# Autodesk Inventor assembly: Shooter Curve Assembly
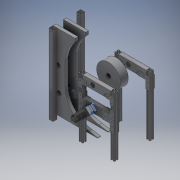
[picture p0: Inventor's stored thumbnail of the model, 180x180]
Saved by Autodesk Inventor 2018 (Build 220112000, 112)
## iProperties
Created: 2020-02-01
Part Number: Shooter Curve Assembly
Document SubType Name: Assembly
Designer: Weeb No1
Author: Weeb No1
## Documents named in this file (13)
- C:\Users\T3500STATIC\Documents\GitHub\2020CAD\Gabriel Inventor Files (Shooter, Drivebase)\V2 Shooter Curve Assembly\Main Assembly File\V2 Shooter Curve Assembly.iam
- C:\Users\T3500STATIC\Documents\GitHub\2020CAD\Gabriel Inventor Files (Shooter, Drivebase)\V2 Shooter Curve Assembly\Part Files\8020 1010 x 15.ipt
- C:\Users\T3500STATIC\Documents\GitHub\2020CAD\Gabriel Inventor Files (Shooter, Drivebase)\V2 Shooter Curve Assembly\Part Files\1x2 5 in Beam Flywheel Mount.ipt
- C:\Users\T3500STATIC\Documents\GitHub\2020CAD\Over bumper intake\Parts\VersaPlanetary_v2_Single_Stage_10_1_with_775_Series.iam
- C:\Users\T3500STATIC\Documents\GitHub\2020CAD\Gabriel Inventor Files (Shooter, Drivebase)\V2 Shooter Curve Assembly\Part Files\1x2 7 in Beam Motor Mount.ipt
- C:\Users\T3500STATIC\Documents\GitHub\2020CAD\Gabriel Inventor Files (Shooter, Drivebase)\Gussets\L-Gusset 3 Hole 0.25in Hole.ipt
- C:\Users\T3500STATIC\Documents\GitHub\2020CAD\Gabriel Inventor Files (Shooter, Drivebase)\V2 Shooter Curve Assembly\Part Files\1x1 20 in Curve Support Beam.ipt
- C:\Users\T3500STATIC\Documents\GitHub\2020CAD\Gabriel Inventor Files (Shooter, Drivebase)\Gussets\L-Guesset 4 Hole 0.25in Hole.ipt
- C:\Users\T3500STATIC\Documents\GitHub\2020CAD\Gabriel Inventor Files (Shooter, Drivebase)\Gussets\L-Guesset 5 Hole 0.25in Hole.ipt
- C:\Users\T3500STATIC\Documents\GitHub\2020CAD\Gabriel Inventor Files (Shooter, Drivebase)\V2 Shooter Curve Assembly\Part Files\_18t_Aluminum_Hub_Sprocket_25_Chain_1_2_Hex_Bore_217-3488.ipt
- C:\Users\T3500STATIC\Documents\GitHub\2020CAD\Gabriel Inventor Files (Shooter, Drivebase)\V2 Shooter Curve Assembly\Part Files\2_OD_Straight_Flex_Wheel_217-6354.ipt
- C:\Users\T3500STATIC\Documents\GitHub\2020CAD\Gabriel Inventor Files (Shooter, Drivebase)\V2 Shooter Curve Assembly\Part Files\New Shooter Curve.ipt
- C:\Users\T3500STATIC\Documents\GitHub\2020CAD\Gabriel Inventor Files (Shooter, Drivebase)\V2 Shooter Curve Assembly\Part Files\Pretend it's a Flywheel.ipt
## Components (33 placed, 12 different names)
1. 8020 1010 x 15:1 — Flush:5, Flush:6, Mate:7, Flush:11, Flush:14, Flush:23, Flush:24, Mate:51, Mate:56, Mate:60, Mate:82, Mate:85, Mate:97, Mate:100, Flush:45, Flush:48, Flush:52
2. 8020 1010 x 15:2 — Flush:7, Mate:9, Flush:15, Flush:22, Flush:25, Mate:127, Mate:130, Flush:44, Flush:46, Flush:51
3. 8020 1010 x 15:3 — Flush:5, Flush:6, Flush:10, Flush:12, Flush:13, Mate:11, Flush:23, Mate:50, Flush:34, Mate:63, Mate:65, Mate:89, Mate:93, Mate:103, Mate:123, Flush:49
4. 8020 1010 x 15:4 — Flush:7, Flush:10, Flush:17, Mate:10, Flush:22, Mate:107, Mate:111, Flush:47
5. 1x2 5 in Beam Flywheel Mount:1 — Mate:9, Flush:15, Flush:17, Mate:10, Flush:25, Mate:106, Mate:108, Mate:109, Mate:110, Mate:112, Mate:113, Mate:126, Mate:128, Mate:129, Mate:131, Mate:137, Flush:50, Mate:138, Mate:140
6. 1x2 5 in Beam Flywheel Mount:2 — Mate:7, Flush:11, Flush:12, Flush:13, Flush:14, Mate:11, Flush:24, Mate:55, Mate:57, Mate:58, Mate:59, Mate:61, Mate:62, Mate:64, Mate:66, Mate:137, Flush:50, Mate:139, Mate:141
7. VersaPlanetary_v2_Single_Stage_10_1_with_775_Series:1 [sub-assembly] — Mate:52, Mate:53, Mate:54
8. 1x2 7 in Beam Motor Mount:1 — Mate:50, Mate:51, Flush:34, Mate:52, Mate:53, Mate:54, Mate:81, Mate:83, Mate:86, Mate:87, Mate:88, Mate:90, Mate:91, Mate:92, Mate:94, Mate:95, Mate:96, Mate:98, Mate:99, Mate:101, Mate:102, Mate:104, Mate:105, Mate:122, Mate:124, Mate:125
9. L-Gusset 3 Hole 0.25in Hole:1 — Mate:61, Mate:62, Mate:63
10. L-Gusset 3 Hole 0.25in Hole:2 — Mate:55, Mate:56, Mate:57
11. L-Gusset 3 Hole 0.25in Hole:3 — Mate:58, Mate:59, Mate:60
12. L-Gusset 3 Hole 0.25in Hole:4 — Mate:64, Mate:65, Mate:66
13. 1x1 20 in Curve Support Beam:1 — Mate:132, Flush:35, Flush:36, Flush:40, Flush:41, Flush:45, Flush:52
14. 1x1 20 in Curve Support Beam:2 — Mate:133, Flush:37, Flush:38, Flush:39, Flush:41, Flush:44, Flush:51
15. L-Guesset 4 Hole 0.25in Hole:3 — Mate:88, Mate:89, Mate:90, Mate:91
16. L-Guesset 4 Hole 0.25in Hole:5 — Mate:81, Mate:82, Mate:83
17. L-Guesset 4 Hole 0.25in Hole:6 — Mate:85, Mate:86, Mate:87
18. L-Guesset 4 Hole 0.25in Hole:9 — Mate:92, Mate:93, Mate:94, Mate:95
19. L-Gusset 3 Hole 0.25in Hole:9 — Mate:96, Mate:97, Mate:98
20. L-Gusset 3 Hole 0.25in Hole:10 — Mate:99, Mate:100, Mate:101
21. L-Guesset 5 Hole 0.25in Hole:1 — Mate:102, Mate:103, Mate:104, Mate:105
22. L-Guesset 5 Hole 0.25in Hole:2 — Mate:110, Mate:111, Mate:112, Mate:113
23. L-Guesset 5 Hole 0.25in Hole:3 — Mate:106, Mate:107, Mate:108, Mate:109
24. L-Guesset 5 Hole 0.25in Hole:6 — Mate:122, Mate:123, Mate:124, Mate:125
25. L-Gusset 3 Hole 0.25in Hole:11 — Mate:126, Mate:127, Mate:128
26. L-Gusset 3 Hole 0.25in Hole:12 — Mate:129, Mate:130, Mate:131
27. _18t_Aluminum_Hub_Sprocket_25_Chain_1_2_Hex_Bore_217-3488:1
28. 2_OD_Straight_Flex_Wheel_217-6354:1
29. 2_OD_Straight_Flex_Wheel_217-6354:2
30. New Shooter Curve:1 — Mate:132, Flush:35, Flush:36, Flush:40, Mate:135, Mate:136, Flush:42, Flush:43, Flush:48, Flush:49, Flush:53, Flush:55
31. New Shooter Curve:2 — Mate:134, Mate:135, Flush:53, Flush:54, Flush:55, Flush:56
32. New Shooter Curve:3 — Mate:133, Flush:37, Flush:38, Flush:39, Mate:134, Mate:136, Flush:42, Flush:43, Flush:46, Flush:47, Flush:54, Flush:56
33. Pretend it's a Flywheel:1 — Mate:138, Mate:139, Mate:140, Mate:141
## Relationships (110: Mate 73, Flush 37)
- Flush:5: 8020 1010 x 15:1 ↔ 8020 1010 x 15:3
- Flush:6: 8020 1010 x 15:1 ↔ 8020 1010 x 15:3
- Flush:7: 8020 1010 x 15:2 ↔ 8020 1010 x 15:4
- Flush:10: 8020 1010 x 15:3 ↔ 8020 1010 x 15:4
- Mate:7: 8020 1010 x 15:1 ↔ 1x2 5 in Beam Flywheel Mount:2
- Flush:11: 8020 1010 x 15:1 ↔ 1x2 5 in Beam Flywheel Mount:2
- Flush:12: 8020 1010 x 15:3 ↔ 1x2 5 in Beam Flywheel Mount:2
- Flush:13: 8020 1010 x 15:3 ↔ 1x2 5 in Beam Flywheel Mount:2
- Flush:14: 8020 1010 x 15:1 ↔ 1x2 5 in Beam Flywheel Mount:2
- Mate:9: 8020 1010 x 15:2 ↔ 1x2 5 in Beam Flywheel Mount:1
- Flush:15: 8020 1010 x 15:2 ↔ 1x2 5 in Beam Flywheel Mount:1
- Flush:17: 8020 1010 x 15:4 ↔ 1x2 5 in Beam Flywheel Mount:1
- Mate:10: 8020 1010 x 15:4 ↔ 1x2 5 in Beam Flywheel Mount:1
- Mate:11: 8020 1010 x 15:3 ↔ 1x2 5 in Beam Flywheel Mount:2
- Flush:22: 8020 1010 x 15:2 ↔ 8020 1010 x 15:4
- Flush:23: 8020 1010 x 15:1 ↔ 8020 1010 x 15:3
- Flush:24: 8020 1010 x 15:1 ↔ 1x2 5 in Beam Flywheel Mount:2
- Flush:25: 8020 1010 x 15:2 ↔ 1x2 5 in Beam Flywheel Mount:1
- Mate:50: 8020 1010 x 15:3 ↔ 1x2 7 in Beam Motor Mount:1
- Mate:51: 8020 1010 x 15:1 ↔ 1x2 7 in Beam Motor Mount:1
- Flush:34: 8020 1010 x 15:3 ↔ 1x2 7 in Beam Motor Mount:1
- Mate:52: VersaPlanetary_v2_Single_Stage_10_1_with_775_Series:1 ↔ 1x2 7 in Beam Motor Mount:1
- Mate:53: VersaPlanetary_v2_Single_Stage_10_1_with_775_Series:1 ↔ 1x2 7 in Beam Motor Mount:1
- Mate:54: VersaPlanetary_v2_Single_Stage_10_1_with_775_Series:1 ↔ 1x2 7 in Beam Motor Mount:1
- Mate:55: 1x2 5 in Beam Flywheel Mount:2 ↔ L-Gusset 3 Hole 0.25in Hole:2
- Mate:56: 8020 1010 x 15:1 ↔ L-Gusset 3 Hole 0.25in Hole:2
- Mate:57: 1x2 5 in Beam Flywheel Mount:2 ↔ L-Gusset 3 Hole 0.25in Hole:2
- Mate:58: 1x2 5 in Beam Flywheel Mount:2 ↔ L-Gusset 3 Hole 0.25in Hole:3
- Mate:59: 1x2 5 in Beam Flywheel Mount:2 ↔ L-Gusset 3 Hole 0.25in Hole:3
- Mate:60: 8020 1010 x 15:1 ↔ L-Gusset 3 Hole 0.25in Hole:3
- Mate:61: 1x2 5 in Beam Flywheel Mount:2 ↔ L-Gusset 3 Hole 0.25in Hole:1
- Mate:62: 1x2 5 in Beam Flywheel Mount:2 ↔ L-Gusset 3 Hole 0.25in Hole:1
- Mate:63: 8020 1010 x 15:3 ↔ L-Gusset 3 Hole 0.25in Hole:1
- Mate:64: 1x2 5 in Beam Flywheel Mount:2 ↔ L-Gusset 3 Hole 0.25in Hole:4
- Mate:65: 8020 1010 x 15:3 ↔ L-Gusset 3 Hole 0.25in Hole:4
- Mate:66: 1x2 5 in Beam Flywheel Mount:2 ↔ L-Gusset 3 Hole 0.25in Hole:4
- Mate:81: 1x2 7 in Beam Motor Mount:1 ↔ L-Guesset 4 Hole 0.25in Hole:5
- Mate:82: 8020 1010 x 15:1 ↔ L-Guesset 4 Hole 0.25in Hole:5
- Mate:83: 1x2 7 in Beam Motor Mount:1 ↔ L-Guesset 4 Hole 0.25in Hole:5
- Mate:85: 8020 1010 x 15:1 ↔ L-Guesset 4 Hole 0.25in Hole:6
- Mate:86: 1x2 7 in Beam Motor Mount:1 ↔ L-Guesset 4 Hole 0.25in Hole:6
- Mate:87: 1x2 7 in Beam Motor Mount:1 ↔ L-Guesset 4 Hole 0.25in Hole:6
- Mate:88: 1x2 7 in Beam Motor Mount:1 ↔ L-Guesset 4 Hole 0.25in Hole:3
- Mate:89: 8020 1010 x 15:3 ↔ L-Guesset 4 Hole 0.25in Hole:3
- Mate:90: 1x2 7 in Beam Motor Mount:1 ↔ L-Guesset 4 Hole 0.25in Hole:3
- Mate:91: 1x2 7 in Beam Motor Mount:1 ↔ L-Guesset 4 Hole 0.25in Hole:3
- Mate:92: 1x2 7 in Beam Motor Mount:1 ↔ L-Guesset 4 Hole 0.25in Hole:9
- Mate:93: 8020 1010 x 15:3 ↔ L-Guesset 4 Hole 0.25in Hole:9
- Mate:94: 1x2 7 in Beam Motor Mount:1 ↔ L-Guesset 4 Hole 0.25in Hole:9
- Mate:95: 1x2 7 in Beam Motor Mount:1 ↔ L-Guesset 4 Hole 0.25in Hole:9
- Mate:96: 1x2 7 in Beam Motor Mount:1 ↔ L-Gusset 3 Hole 0.25in Hole:9
- Mate:97: 8020 1010 x 15:1 ↔ L-Gusset 3 Hole 0.25in Hole:9
- Mate:98: 1x2 7 in Beam Motor Mount:1 ↔ L-Gusset 3 Hole 0.25in Hole:9
- Mate:99: 1x2 7 in Beam Motor Mount:1 ↔ L-Gusset 3 Hole 0.25in Hole:10
- Mate:100: 8020 1010 x 15:1 ↔ L-Gusset 3 Hole 0.25in Hole:10
- Mate:101: 1x2 7 in Beam Motor Mount:1 ↔ L-Gusset 3 Hole 0.25in Hole:10
- Mate:102: 1x2 7 in Beam Motor Mount:1 ↔ L-Guesset 5 Hole 0.25in Hole:1
- Mate:103: 8020 1010 x 15:3 ↔ L-Guesset 5 Hole 0.25in Hole:1
- Mate:104: 1x2 7 in Beam Motor Mount:1 ↔ L-Guesset 5 Hole 0.25in Hole:1
- Mate:105: 1x2 7 in Beam Motor Mount:1 ↔ L-Guesset 5 Hole 0.25in Hole:1
- Mate:106: 1x2 5 in Beam Flywheel Mount:1 ↔ L-Guesset 5 Hole 0.25in Hole:3
- Mate:107: 8020 1010 x 15:4 ↔ L-Guesset 5 Hole 0.25in Hole:3
- Mate:108: 1x2 5 in Beam Flywheel Mount:1 ↔ L-Guesset 5 Hole 0.25in Hole:3
- Mate:109: 1x2 5 in Beam Flywheel Mount:1 ↔ L-Guesset 5 Hole 0.25in Hole:3
- Mate:110: 1x2 5 in Beam Flywheel Mount:1 ↔ L-Guesset 5 Hole 0.25in Hole:2
- Mate:111: 8020 1010 x 15:4 ↔ L-Guesset 5 Hole 0.25in Hole:2
- Mate:112: 1x2 5 in Beam Flywheel Mount:1 ↔ L-Guesset 5 Hole 0.25in Hole:2
- Mate:113: 1x2 5 in Beam Flywheel Mount:1 ↔ L-Guesset 5 Hole 0.25in Hole:2
- Mate:122: 1x2 7 in Beam Motor Mount:1 ↔ L-Guesset 5 Hole 0.25in Hole:6
- Mate:123: 8020 1010 x 15:3 ↔ L-Guesset 5 Hole 0.25in Hole:6
- Mate:124: 1x2 7 in Beam Motor Mount:1 ↔ L-Guesset 5 Hole 0.25in Hole:6
- Mate:125: 1x2 7 in Beam Motor Mount:1 ↔ L-Guesset 5 Hole 0.25in Hole:6
- Mate:126: 1x2 5 in Beam Flywheel Mount:1 ↔ L-Gusset 3 Hole 0.25in Hole:11
- Mate:127: 8020 1010 x 15:2 ↔ L-Gusset 3 Hole 0.25in Hole:11
- Mate:128: 1x2 5 in Beam Flywheel Mount:1 ↔ L-Gusset 3 Hole 0.25in Hole:11
- Mate:129: 1x2 5 in Beam Flywheel Mount:1 ↔ L-Gusset 3 Hole 0.25in Hole:12
- Mate:130: 8020 1010 x 15:2 ↔ L-Gusset 3 Hole 0.25in Hole:12
- Mate:131: 1x2 5 in Beam Flywheel Mount:1 ↔ L-Gusset 3 Hole 0.25in Hole:12
- Mate:132: 1x1 20 in Curve Support Beam:1 ↔ New Shooter Curve:1
- Flush:35: 1x1 20 in Curve Support Beam:1 ↔ New Shooter Curve:1
- Flush:36 (25.4 mm): 1x1 20 in Curve Support Beam:1 ↔ New Shooter Curve:1
- Mate:133: 1x1 20 in Curve Support Beam:2 ↔ New Shooter Curve:3
- Flush:37: 1x1 20 in Curve Support Beam:2 ↔ New Shooter Curve:3
- Flush:38 (25.4 mm): 1x1 20 in Curve Support Beam:2 ↔ New Shooter Curve:3
- Flush:39: 1x1 20 in Curve Support Beam:2 ↔ New Shooter Curve:3
- Flush:40: 1x1 20 in Curve Support Beam:1 ↔ New Shooter Curve:1
- Mate:134 (47.625 mm): New Shooter Curve:2 ↔ New Shooter Curve:3
- Mate:135 (47.625 mm): New Shooter Curve:1 ↔ New Shooter Curve:2
- Mate:136 (114.3 mm): New Shooter Curve:1 ↔ New Shooter Curve:3
- Flush:41: 1x1 20 in Curve Support Beam:1 ↔ 1x1 20 in Curve Support Beam:2
- Flush:42: New Shooter Curve:1 ↔ New Shooter Curve:3
- Flush:43: New Shooter Curve:1 ↔ New Shooter Curve:3
- Flush:44 (215.9 mm): 8020 1010 x 15:2 ↔ 1x1 20 in Curve Support Beam:2
- Flush:45 (215.9 mm): 8020 1010 x 15:1 ↔ 1x1 20 in Curve Support Beam:1
- Flush:46 (-25.4 mm): 8020 1010 x 15:2 ↔ New Shooter Curve:3
- Flush:47 (-25.4 mm): 8020 1010 x 15:4 ↔ New Shooter Curve:3
- Flush:48 (-25.4 mm): 8020 1010 x 15:1 ↔ New Shooter Curve:1
- Flush:49 (-25.4 mm): 8020 1010 x 15:3 ↔ New Shooter Curve:1
- Mate:137 (203.2 mm): 1x2 5 in Beam Flywheel Mount:1 ↔ 1x2 5 in Beam Flywheel Mount:2
- Flush:50: 1x2 5 in Beam Flywheel Mount:1 ↔ 1x2 5 in Beam Flywheel Mount:2
- Flush:51 (-25.4 mm): 8020 1010 x 15:2 ↔ 1x1 20 in Curve Support Beam:2
- Flush:52 (-25.4 mm): 8020 1010 x 15:1 ↔ 1x1 20 in Curve Support Beam:1
- Mate:138 (76.2 mm): 1x2 5 in Beam Flywheel Mount:1 ↔ Pretend it's a Flywheel:1
- Mate:139 (76.2 mm): 1x2 5 in Beam Flywheel Mount:2 ↔ Pretend it's a Flywheel:1
- Mate:140: 1x2 5 in Beam Flywheel Mount:1 ↔ Pretend it's a Flywheel:1
- Mate:141: 1x2 5 in Beam Flywheel Mount:2 ↔ Pretend it's a Flywheel:1
- Flush:53: New Shooter Curve:1 ↔ New Shooter Curve:2
- Flush:54: New Shooter Curve:2 ↔ New Shooter Curve:3
- Flush:55: New Shooter Curve:1 ↔ New Shooter Curve:2
- Flush:56: New Shooter Curve:2 ↔ New Shooter Curve:3
